# Autodesk Inventor assembly: payload mount
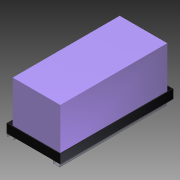
[picture p0: Inventor's stored thumbnail of the model, 180x180]
Saved by Autodesk Inventor 2012 (Build 160160000, 160)
## iProperties
Created: 2011-12-02
Part Number: payload mount
Document SubType Name: Assembly
Designer: Antonella
Author: Antonella
## Documents named in this file (4)
- C:\Users\Antonella\Documents\GCC Robotics 2012 - Mechanical\Robot 2.0\Payload Mount\payload mount.iam
- C:\Users\Antonella\Documents\GCC Robotics 2012 - Mechanical\Robot 2.0\Payload Mount\slide.iam
- C:\Users\Antonella\Documents\GCC Robotics 2012 - Mechanical\Robot 2.0\Payload Mount\tray.iam
- C:\Users\Antonella\Documents\GCC Robotics 2012 - Mechanical\Robot 2.0\Payload Mount\payload.ipt
## Components (4 placed, 3 different names)
1. tray:1 [sub-assembly] — Mate:1, Mate:2, Tangent:1, Tangent:2, Mate:3, Mate:4, Flush:3, Flush:5, Flush:6
2. slide:1 [sub-assembly] — Mate:1, Tangent:2, Flush:5
3. slide:2 [sub-assembly] — Mate:2, Tangent:1, Flush:6
4. payload:1 — Mate:3, Mate:4, Flush:3
## Relationships (9: Mate 4, Flush 3, Tangent 2)
- Mate:1: tray:1 ↔ slide:1
- Mate:2: tray:1 ↔ slide:2
- Tangent:1: tray:1 ↔ slide:2
- Tangent:2: tray:1 ↔ slide:1
- Mate:3: tray:1 ↔ payload:1
- Mate:4: tray:1 ↔ payload:1
- Flush:3: tray:1 ↔ payload:1
- Flush:5: tray:1 ↔ slide:1
- Flush:6: tray:1 ↔ slide:2
